# Autodesk Inventor assembly: FINISHEDASSEMBLY
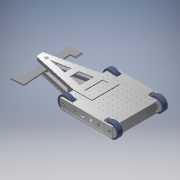
[picture p0: Inventor's stored thumbnail of the model, 180x180]
Saved by Autodesk Inventor 2017 (Build 210142000, 142)
## iProperties
Created: 2016-11-05
Part Number: FINISHEDASSEMBLY
Document SubType Name: Assembly
Designer: Kevin G
Author: Kevin G
## Documents named in this file (6)
- C:\Users\aesen\Design\newassembly\ASSEMBLY-W1.iam
- C:\Users\aesen\Design\newassembly\NEWDRIVETRAINBOXWITHGEARS.iam
- C:\Users\aesen\Design\newassembly\1023TopP.ipt
- C:\Users\aesen\Design\newassembly\FrontPlate.ipt
- C:\Users\aesen\Design\newassembly\Back Plate.ipt
- C:\Users\aesen\Design\newassembly\WPS.iam
## Components (7 placed, 5 different names)
1. NEWDRIVETRAINBOXWITHGEARS:1 [sub-assembly] — Mate:1, Mate:2, Mate:3, Mate:10, Mate:11
2. 1023TopP:1 — Mate:1, Mate:2, Mate:3, Mate:4, Mate:5, Mate:6, Mate:7, Mate:15
3. NEWDRIVETRAINBOXWITHGEARS:2 [sub-assembly] — Mate:4, Mate:5, Mate:6, Mate:7, Mate:8, Mate:9, Mate:13
4. 1023TopP:2 — Mate:8, Mate:9, Mate:10, Mate:12, Mate:14
5. FrontPlate:1 — Mate:11, Mate:12
6. Back Plate:1 — Mate:13, Mate:14
7. WPS:1 [sub-assembly] — Mate:15
## Relationships (15: Mate 15)
- Mate:1: NEWDRIVETRAINBOXWITHGEARS:1 ↔ 1023TopP:1
- Mate:2: NEWDRIVETRAINBOXWITHGEARS:1 ↔ 1023TopP:1
- Mate:3: NEWDRIVETRAINBOXWITHGEARS:1 ↔ 1023TopP:1
- Mate:4: 1023TopP:1 ↔ NEWDRIVETRAINBOXWITHGEARS:2
- Mate:5: 1023TopP:1 ↔ NEWDRIVETRAINBOXWITHGEARS:2
- Mate:6: 1023TopP:1 ↔ NEWDRIVETRAINBOXWITHGEARS:2
- Mate:7: 1023TopP:1 ↔ NEWDRIVETRAINBOXWITHGEARS:2
- Mate:8: NEWDRIVETRAINBOXWITHGEARS:2 ↔ 1023TopP:2
- Mate:9: NEWDRIVETRAINBOXWITHGEARS:2 ↔ 1023TopP:2
- Mate:10: NEWDRIVETRAINBOXWITHGEARS:1 ↔ 1023TopP:2
- Mate:11: NEWDRIVETRAINBOXWITHGEARS:1 ↔ FrontPlate:1
- Mate:12: 1023TopP:2 ↔ FrontPlate:1
- Mate:13: NEWDRIVETRAINBOXWITHGEARS:2 ↔ Back Plate:1
- Mate:14: 1023TopP:2 ↔ Back Plate:1
- Mate:15: 1023TopP:1 ↔ WPS:1
